# Autodesk Inventor assembly: funnel_back
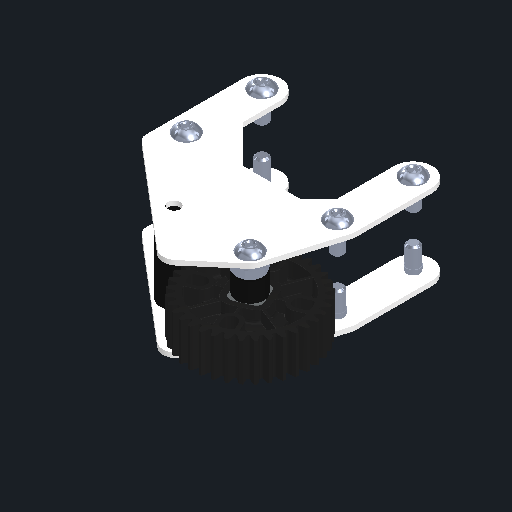
[picture p0: Inventor's stored thumbnail of the model, 512x512]
Saved by Autodesk Inventor 2025 (Build 290162000, 162)
## iProperties
Created: 2024-10-04
Part Number: funnel_back
Document SubType Name: Assembly
Designer: Averey Ku
Author: Averey Ku
## Documents named in this file (17)
- D:\vex_robotics_high_stakes\hardware\cad\bots\high_stakes_v2\chassis\drivebay\funnel_back.iam
- D:\vex_robotics_high_stakes\hardware\cad\bots\high_stakes_v2\chassis\drivebay\custom_parts\gusset.ipt
- D:\vex_robotics_high_stakes\hardware\cad\robpros_cad_lib\Motion\Spacers\Washer Steel\SWasher .375 OD x .062500.ipt
- D:\vex_robotics_high_stakes\hardware\cad\robpros_cad_lib\Motion\Spacers\Washer Steel.ipt
- D:\vex_robotics_high_stakes\hardware\cad\robpros_cad_lib\Structure\Hardware\Nut Keps.ipt
- D:\vex_robotics_high_stakes\hardware\cad\robpros_cad_lib\Motion\Spacers\Spacer Nylon .375 OD\NSpacer .375 OD x .250.ipt
- D:\vex_robotics_high_stakes\hardware\cad\robpros_cad_lib\Motion\Spacers\Spacer Nylon .375 OD.ipt
- D:\vex_robotics_high_stakes\hardware\cad\robpros_cad_lib\Motion\Spacers\Washer Steel\SWasher .375 OD x .031250.ipt
- D:\vex_robotics_high_stakes\hardware\cad\VEX-CAD-Inventor\Structure\Hardware\Screw Steel - Star\SScrew Star Smooth .250.ipt
- D:\vex_robotics_high_stakes\hardware\cad\VEX-CAD-Inventor\Structure\Hardware\Screw Steel - Star.ipt
- D:\vex_robotics_high_stakes\hardware\cad\VEX-CAD-Inventor\Structure\Hardware\Screw Steel - Star\SScrew Star Smooth 1.250.ipt
- D:\vex_robotics_high_stakes\hardware\cad\VEX-CAD-Inventor\Structure\Hardware\Nut Hex.ipt
- D:\vex_robotics_high_stakes\hardware\cad\VEX-CAD-Inventor\Structure\Hardware\Screw Shoulder Robosource\SScrew Shoulder Smooth .375 x .12.ipt
- D:\vex_robotics_high_stakes\hardware\cad\VEX-CAD-Inventor\Structure\Hardware\Screw Shoulder Robosource.ipt
- D:\vex_robotics_high_stakes\hardware\cad\robpros_cad_lib\Motion\Spacers\Spacer Nylon .375 OD\NSpacer .375 OD x .500.ipt
- D:\vex_robotics_high_stakes\hardware\cad\robpros_cad_lib\Motion\Gears\HS Gear\HS 36T Gear, No Insert.iam
- D:\vex_robotics_high_stakes\hardware\cad\robpros_cad_lib\Motion\Gears\HS Gear.iam
## Components (20 placed, 11 different names)
1. gusset:1 — Insert:2, Mate:2, Insert:14, Insert:16, Insert:20, Insert:27
2. gusset:2 — Mate:1, Insert:2, Mate:2, Insert:11, Angle:1, Insert:15, Insert:19
3. SWasher .375 OD x .062500:1 — Insert:9
4. Nut Keps:1 — Insert:7, Insert:16
5. NSpacer .375 OD x .250:1 — Insert:7, Insert:25
6. SWasher .375 OD x .031250:2 — Insert:9
7. SScrew Star Smooth .250:2 — Insert:11
8. SScrew Star Smooth 1.250:3 — Insert:20
9. Nut Hex:1 — Insert:19
10. HS 36T Gear, No Insert:3 [sub-assembly] — Insert:25
11. NSpacer .375 OD x .500:2 — Insert:26
12. NSpacer .375 OD x .500:3 — Insert:26, Insert:27
13. SScrew Shoulder Smooth .375 x .12:1 — Insert:14
14. SScrew Shoulder Smooth .375 x .12:2
15. SScrew Shoulder Smooth .375 x .12:3
16. SScrew Shoulder Smooth .375 x .12:4
17. SScrew Shoulder Smooth .375 x .12:5 — Insert:15
18. SScrew Shoulder Smooth .375 x .12:6
19. SScrew Shoulder Smooth .375 x .12:7
20. SScrew Shoulder Smooth .375 x .12:8
## Component patterns: (4 elements, first: SScrew Shoulder Smooth .375 x .12:1), (4 elements, first: SScrew Shoulder Smooth .375 x .12:5)
## Relationships (15: Insert 12, Mate 2, Angle 1)
- Mate:1: gusset:2
- Insert:2 (25.4 mm): gusset:1 ↔ gusset:2
- Mate:2: gusset:1 ↔ gusset:2
- Insert:7: Nut Keps:1 ↔ NSpacer .375 OD x .250:1
- Insert:9: SWasher .375 OD x .062500:1 ↔ SWasher .375 OD x .031250:2
- Insert:11: gusset:2 ↔ SScrew Star Smooth .250:2
- Insert:14: gusset:1 ↔ SScrew Shoulder Smooth .375 x .12:1
- Angle:1 (0 deg): gusset:2
- Insert:15: gusset:2 ↔ SScrew Shoulder Smooth .375 x .12:5
- Insert:16: gusset:1 ↔ Nut Keps:1
- Insert:19: gusset:2 ↔ Nut Hex:1
- Insert:20: gusset:1 ↔ SScrew Star Smooth 1.250:3
- Insert:25: NSpacer .375 OD x .250:1 ↔ HS 36T Gear, No Insert:3
- Insert:26: NSpacer .375 OD x .500:2 ↔ NSpacer .375 OD x .500:3
- Insert:27: gusset:1 ↔ NSpacer .375 OD x .500:3
